# Autodesk Inventor assembly: MGN7 Rail 150mm (3)
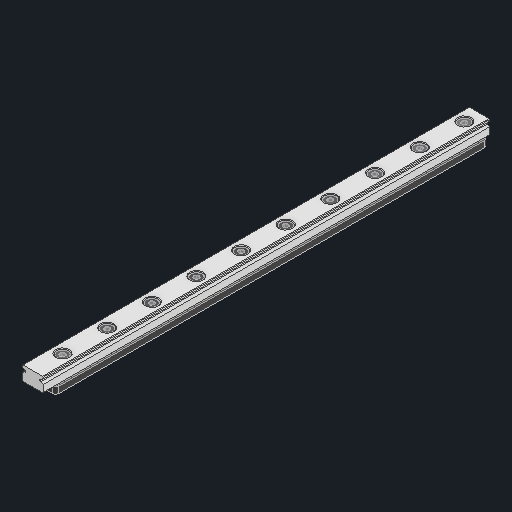
[picture p0: Inventor's stored thumbnail of the model, 512x512]
Saved by Autodesk Inventor 2025.1 (Build 291241020, 241B)
## iProperties
Created: 2025-05-09
Part Number: MGN7 Rail 150mm (3)
Document SubType Name: Assembly
Designer: AdminForWorker
Title: MGN7 150mm Rail
Author: AdminForWorker
## Documents named in this file (5)
- C:\Users\Joshua Eah\Documents\Voron 0.2\CAD\Master Assembly\Linear Rail\MGN7 Rail 150mm.iam
- MGN7 150mm Rail.iam
- C:\Users\Joshua Eah\Documents\Voron 0.2\CAD\Master Assembly\Hardware\M2x6 SHCS.ipt
- C:\Users\Joshua Eah\Documents\Voron 0.2\CAD\Master Assembly\Linear Rail\Parts\150 mm Rail.ipt
- C:\Users\Joshua Eah\Documents\Voron 0.2\CAD\Master Assembly\Linear Rail\Subassemblies\M2 Hex Nuts.iam
## Components (12 placed, 3 different names)
1. 150mm Rail — Insert:1, Insert:2, Insert:3, Insert:4, Insert:5, Insert:6, Insert:7, Insert:8, Insert:9, Insert:10
2. M2x6 SHCS:1 — Insert:1, Insert:11
3. M2x6 SHCS:2 — Insert:6
4. M2x6 SHCS:3 — Insert:2
5. M2x6 SHCS:4 — Insert:9
6. M2x6 SHCS:5 — Insert:8
7. M2x6 SHCS:6 — Insert:4
8. M2x6 SHCS:7 — Insert:3
9. M2x6 SHCS:8 — Insert:7
10. M2x6 SHCS:9 — Insert:10, Insert:12
11. M2x6 SHCS:10 — Insert:5
12. M2 Hex Nuts:1 [sub-assembly] — Insert:11, Insert:12
## Relationships (12: Insert 12)
- Insert:1: 150mm Rail ↔ M2x6 SHCS:1
- Insert:2: 150mm Rail ↔ M2x6 SHCS:3
- Insert:3: 150mm Rail ↔ M2x6 SHCS:7
- Insert:4: 150mm Rail ↔ M2x6 SHCS:6
- Insert:5: 150mm Rail ↔ M2x6 SHCS:10
- Insert:6: 150mm Rail ↔ M2x6 SHCS:2
- Insert:7: 150mm Rail ↔ M2x6 SHCS:8
- Insert:8: 150mm Rail ↔ M2x6 SHCS:5
- Insert:9: 150mm Rail ↔ M2x6 SHCS:4
- Insert:10: 150mm Rail ↔ M2x6 SHCS:9
- Insert:11: M2x6 SHCS:1 ↔ M2 Hex Nuts:1
- Insert:12: M2x6 SHCS:9 ↔ M2 Hex Nuts:1
